# Autodesk Inventor assembly: Slope_HighEnd-FM
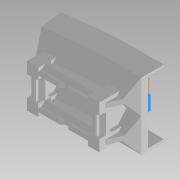
[picture p0: Inventor's stored thumbnail of the model, 180x180]
Saved by Autodesk Inventor 2021 (Build 250183000, 183)
## iProperties
Created: 2021-03-11
Part Number: Slope_HighEnd-FM
Document SubType Name: Assembly
Designer: kumagai
Author: kumagai
## Documents named in this file (8)
- X:\Develop\CAD\PlaRails\VPUSlope\Slope_HighEnd.iam
- X:\Develop\CAD\PlaRails\RailJointFemale_filled.ipt
- X:\Develop\CAD\PlaRails\RailJointMale_filled.ipt
- X:\Develop\CAD\PlaRails\VPUSlope\Slope_HighEnd.ipt
- X:\Develop\CAD\PlaRails\ViaductPillarUnit\VPU_EdgeBottom.ipt
- X:\Develop\CAD\PlaRails\GlobalParameter.ipt
- Slope_HighEnd-FF.iam
- Slope_HighEnd-FM.iam
## Components (6 placed, 4 different names)
1. Slope_HighEnd:1 — メイト:1, メイト:2, フラッシュ:1, フラッシュ:2, メイト:3, メイト:4, フラッシュ:5, フラッシュ:6, メイト:6, メイト:7, メイト:8, フラッシュ:7
2. RailJointFemale_filled:1 — メイト:1, フラッシュ:1, メイト:3
3. RailJointMale_filled:1 — メイト:2, フラッシュ:2, メイト:4
4. VPU_EdgeBottom:1 — メイト:5, フラッシュ:3, フラッシュ:4, フラッシュ:5
5. VPU_EdgeBottom:2 — メイト:5, フラッシュ:3, フラッシュ:4, フラッシュ:6, メイト:6
6. RailJointFemale_filled:2 — メイト:7, メイト:8, フラッシュ:7
## Relationships (15: Mate 8, Flush 7)
- メイト:1 [Mate]: Slope_HighEnd:1 ↔ RailJointFemale_filled:1
- メイト:2 [Mate]: Slope_HighEnd:1 ↔ RailJointMale_filled:1
- フラッシュ:1 [Flush]: Slope_HighEnd:1 ↔ RailJointFemale_filled:1
- フラッシュ:2 [Flush]: Slope_HighEnd:1 ↔ RailJointMale_filled:1
- メイト:3 [Mate]: Slope_HighEnd:1 ↔ RailJointFemale_filled:1
- メイト:4 [Mate]: Slope_HighEnd:1 ↔ RailJointMale_filled:1
- メイト:5 [Mate]: VPU_EdgeBottom:1 ↔ VPU_EdgeBottom:2
- フラッシュ:3 [Flush]: VPU_EdgeBottom:1 ↔ VPU_EdgeBottom:2
- フラッシュ:4 [Flush]: VPU_EdgeBottom:1 ↔ VPU_EdgeBottom:2
- フラッシュ:5 [Flush]: Slope_HighEnd:1 ↔ VPU_EdgeBottom:1
- フラッシュ:6 [Flush] (5 mm): Slope_HighEnd:1 ↔ VPU_EdgeBottom:2
- メイト:6 [Mate] (27.8 mm): Slope_HighEnd:1 ↔ VPU_EdgeBottom:2
- メイト:7 [Mate]: Slope_HighEnd:1 ↔ RailJointFemale_filled:2
- メイト:8 [Mate]: Slope_HighEnd:1 ↔ RailJointFemale_filled:2
- フラッシュ:7 [Flush]: Slope_HighEnd:1 ↔ RailJointFemale_filled:2
## Named parameters: RailWidth = 38 mm, ViaductHeight = 66 mm, RailHeight = 8.4 mm, RailDepth = 3.2 mm
